# Autodesk Inventor assembly: 1x15
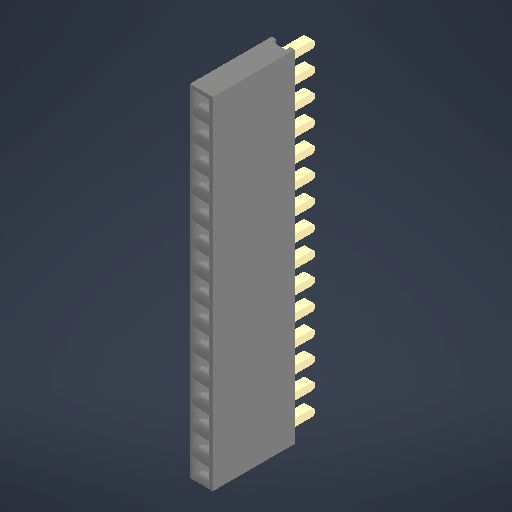
[picture p0: Inventor's stored thumbnail of the model, 512x512]
Saved by Autodesk Inventor 2026.1 (Build 301233020, 233B)
## iProperties
Created: 2026-02-14
Part Number: 1x15
Document SubType Name: Assembly
Designer: celio
Author: celio
## Documents named in this file (3)
- C:\Users\celio\OneDrive\Documentos\Inventor\ZeGuia\Pinos\Femea\1x15\1x15.iam
- C:\Users\celio\OneDrive\Documentos\Inventor\ZeGuia\Pinos\Femea\1x15\parts\1x5.ipt
- C:\Users\celio\OneDrive\Documentos\Inventor\ZeGuia\Pinos\Femea\1x15\parts\1x10.ipt
## Components (2 placed, 2 different names)
1. 1x5:1 — Coincidente:1, Alinhado:1, Alinhado:2
2. 1x10:1 — Coincidente:1, Alinhado:1, Alinhado:2
## Relationships (3: Flush 2, Mate 1)
- Coincidente:1 [Mate]: 1x5:1 ↔ 1x10:1
- Alinhado:1 [Flush]: 1x5:1 ↔ 1x10:1
- Alinhado:2 [Flush]: 1x5:1 ↔ 1x10:1
